# Autodesk Inventor assembly: 112_onering_soro
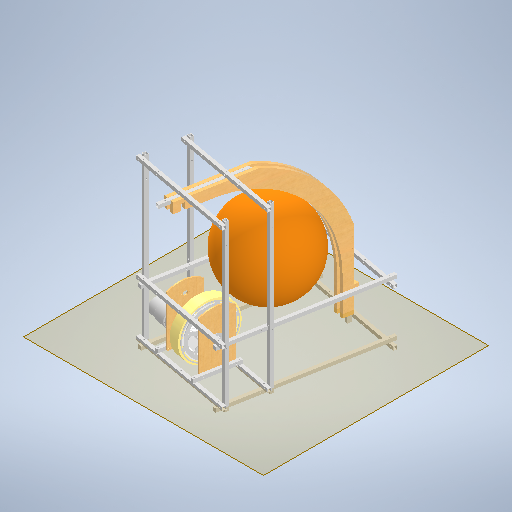
[picture p0: Inventor's stored thumbnail of the model, 512x512]
Saved by Autodesk Inventor 2025.1 (Build 291241000, 241)
## iProperties
Created: 2024-10-08
Part Number: 112_onering_soro
Document SubType Name: Assembly
Designer: yuki0520
Author: yuki0520
## Documents named in this file (4)
- C:\Users\yuki0520\OneDrive\ドキュメント\Inventor\2025_nhk\tanaka\nageru\onering\112_onering_soro.iam
- C:\Users\yuki0520\OneDrive\ドキュメント\Inventor\2025_nhk\tanaka\object\ball.ipt
- C:\Users\yuki0520\OneDrive\ドキュメント\Inventor\2025_nhk\tanaka\nageru\onering\onering_tire_set.iam
- C:\Users\yuki0520\OneDrive\ドキュメント\Inventor\2025_nhk\tanaka\nageru\onering\rail_test_90_nsoro.ipt
## Components (4 placed, 3 different names)
1. ball:1 — 正接:1
2. rail_test_90_nsoro:1 — 挿入:4, 挿入:5, 挿入:6
3. rail_test_90_nsoro:2 — 挿入:1, 挿入:2, 挿入:3, 正接:1
4. onering_tire_set:2 [sub-assembly] — 挿入:1, 挿入:2, 挿入:3, 挿入:4, 挿入:5, 挿入:6
## Relationships (7: Insert 6, Tangent 1)
- 挿入:1 [Insert]: rail_test_90_nsoro:2 ↔ onering_tire_set:2
- 挿入:2 [Insert]: rail_test_90_nsoro:2 ↔ onering_tire_set:2
- 挿入:3 [Insert]: rail_test_90_nsoro:2 ↔ onering_tire_set:2
- 挿入:4 [Insert]: rail_test_90_nsoro:1 ↔ onering_tire_set:2
- 挿入:5 [Insert]: rail_test_90_nsoro:1 ↔ onering_tire_set:2
- 挿入:6 [Insert]: rail_test_90_nsoro:1 ↔ onering_tire_set:2
- 正接:1 [Tangent]: ball:1 ↔ rail_test_90_nsoro:2
